# Autodesk Inventor assembly: Assembly2
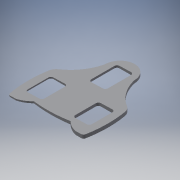
[picture p0: Inventor's stored thumbnail of the model, 180x180]
Saved by Autodesk Inventor 2019 (Build 230136000, 136)
## iProperties
Created: 2019-06-11
Part Number: Assembly2
Document SubType Name: Assembly
Designer: assman
Author: assman
## Documents named in this file (4)
- D:\Inventor\Projects\Calas Carretera\Assembly2.iam
- D:\Inventor\Projects\Calas Carretera\cutaway_1mm.ipt
- D:\Inventor\Projects\Calas Carretera\shim_2_mm.ipt
- D:\Inventor\Projects\Part6.ipt
## Components (3 placed, 3 different names)
1. cutaway_1mm:1 — Rigid:1
2. shim_2_mm:1 — Rigid:1
3. Part6:1
## Relationships (1: WeldJoint 1)
- Rigid:1 [WeldJoint] (-20 mm): cutaway_1mm:1 ↔ shim_2_mm:1
